# Autodesk Inventor assembly: Bartosz_Zukowski_Wycieraczki_zespol
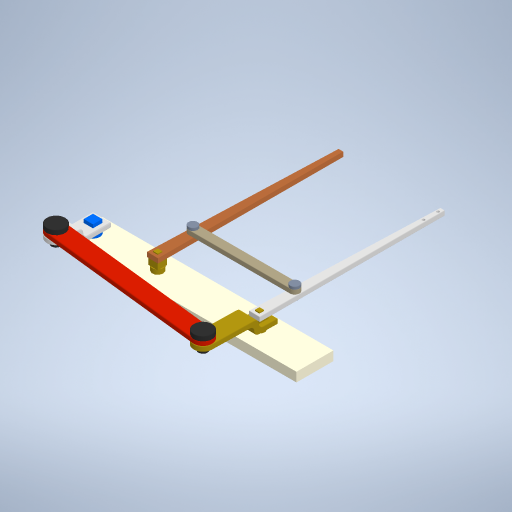
[picture p0: Inventor's stored thumbnail of the model, 512x512]
Saved by Autodesk Inventor 2024 (Build 280153000, 153)
## iProperties
Created: 2024-05-31
Part Number: Bartosz_Zukowski_Wycieraczki_zespol
Document SubType Name: Assembly
Designer: Bartosz
Author: Bartosz
## Documents named in this file (12)
- C:\Users\Barto\Documents\Inventor\Bartosz_Zukowski_IP_2023_2024\Bartosz_Zukowski_Wycieraczki_zespol.iam
- C:\Users\Barto\Documents\Inventor\Bartosz_Zukowski_IP_2023_2024\wycieraczki\podstawa.ipt
- C:\Users\Barto\Documents\Inventor\Bartosz_Zukowski_IP_2023_2024\wycieraczki\sworzeõ napedowy.ipt
- C:\Users\Barto\Documents\Inventor\Bartosz_Zukowski_IP_2023_2024\wycieraczki\sworzen2.ipt
- C:\Users\Barto\Documents\Inventor\Bartosz_Zukowski_IP_2023_2024\wycieraczki\ramie krótkie.ipt
- C:\Users\Barto\Documents\Inventor\Bartosz_Zukowski_IP_2023_2024\wycieraczki\êacznik2.ipt
- C:\Users\Barto\Documents\Inventor\Bartosz_Zukowski_IP_2023_2024\wycieraczki\pióro2.ipt
- C:\Users\Barto\Documents\Inventor\Bartosz_Zukowski_IP_2023_2024\wycieraczki\pióro1.ipt
- C:\Users\Barto\Documents\Inventor\Bartosz_Zukowski_IP_2023_2024\wycieraczki\ramie dêugie.ipt
- C:\Users\Barto\Documents\Inventor\Bartosz_Zukowski_IP_2023_2024\wycieraczki\êÑcznik piór.ipt
- C:\Users\Barto\Documents\Inventor\Bartosz_Zukowski_IP_2023_2024\wycieraczki\sworzen êÑcznikowy 1.ipt
- C:\Users\Barto\Documents\Inventor\Bartosz_Zukowski_IP_2023_2024\wycieraczki\sworzen êÑcznikowy.ipt
## Components (14 placed, 11 different names)
1. podstawa:1 — Wstawiające:1, Wstawiające:2, Wstawiające:3, Kątowe:1
2. sworzeõ napedowy:1 — Wstawiające:1, Zestawiające:1, Zestawiające:2, Zestawiające:3, Kątowe:1
3. sworzen2:1 — Wstawiające:2, Zestawiające:7, Zestawiające:8, Zestawiające:9
4. sworzen2:2 — Wstawiające:3, Zestawiające:4, Zestawiające:5, Zestawiające:6, Zestawiające:10, Zestawiające:11, Zestawiające:18
5. ramie krótkie:1 — Zestawiające:1, Zestawiające:2, Zestawiające:3, Zestawiające:14
6. êacznik2:1 — Zestawiające:4, Zestawiające:5, Zestawiające:6, Zestawiające:12, Zestawiające:13
7. pióro2:1 — Zestawiające:7, Zestawiające:8, Zestawiające:9, Zestawiające:15, Zestawiające:17
8. pióro1:1 — Zestawiające:10, Zestawiające:11, Zestawiające:16, Zestawiające:18
9. ramie dêugie:1 — Zestawiające:12, Zestawiające:13, Zestawiające:14, Wstawiające:6, Wstawiające:7
10. êÑcznik piór:1 — Zestawiające:15, Zestawiające:16, Zestawiające:17, Wstawiające:5, Wstawiające:8
11. sworzen êÑcznikowy 1:1 — Wstawiające:7
12. sworzen êÑcznikowy 1:2 — Wstawiające:6
13. sworzen êÑcznikowy:1 — Wstawiające:5
14. sworzen êÑcznikowy:2 — Wstawiające:8
## Relationships (26: Mate 18, Insert 7, Angle 1)
- Wstawiające:1 [Insert]: podstawa:1 ↔ sworzeõ napedowy:1
- Wstawiające:2 [Insert]: podstawa:1 ↔ sworzen2:1
- Wstawiające:3 [Insert]: podstawa:1 ↔ sworzen2:2
- Zestawiające:1 [Mate]: sworzeõ napedowy:1 ↔ ramie krótkie:1
- Zestawiające:2 [Mate]: sworzeõ napedowy:1 ↔ ramie krótkie:1
- Zestawiające:3 [Mate]: sworzeõ napedowy:1 ↔ ramie krótkie:1
- Zestawiające:4 [Mate]: sworzen2:2 ↔ êacznik2:1
- Zestawiające:5 [Mate]: sworzen2:2 ↔ êacznik2:1
- Zestawiające:6 [Mate]: sworzen2:2 ↔ êacznik2:1
- Zestawiające:7 [Mate]: sworzen2:1 ↔ pióro2:1
- Zestawiające:8 [Mate]: sworzen2:1 ↔ pióro2:1
- Zestawiające:9 [Mate]: sworzen2:1 ↔ pióro2:1
- Zestawiające:10 [Mate]: sworzen2:2 ↔ pióro1:1
- Zestawiające:11 [Mate]: sworzen2:2 ↔ pióro1:1
- Zestawiające:12 [Mate]: êacznik2:1 ↔ ramie dêugie:1
- Zestawiające:13 [Mate]: êacznik2:1 ↔ ramie dêugie:1
- Zestawiające:14 [Mate]: ramie krótkie:1 ↔ ramie dêugie:1
- Zestawiające:15 [Mate]: pióro2:1 ↔ êÑcznik piór:1
- Zestawiające:16 [Mate]: pióro1:1 ↔ êÑcznik piór:1
- Zestawiające:17 [Mate]: pióro2:1 ↔ êÑcznik piór:1
- Zestawiające:18 [Mate]: sworzen2:2 ↔ pióro1:1
- Kątowe:1 [Angle] (360 deg): podstawa:1 ↔ sworzeõ napedowy:1
- Wstawiające:5 [Insert]: êÑcznik piór:1 ↔ sworzen êÑcznikowy:1
- Wstawiające:6 [Insert]: ramie dêugie:1 ↔ sworzen êÑcznikowy 1:2
- Wstawiające:7 [Insert]: ramie dêugie:1 ↔ sworzen êÑcznikowy 1:1
- Wstawiające:8 [Insert]: êÑcznik piór:1 ↔ sworzen êÑcznikowy:2
